# Autodesk Inventor assembly: Assembly1
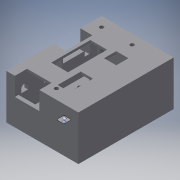
[picture p0: Inventor's stored thumbnail of the model, 180x180]
Saved by Autodesk Inventor 2017 (Build 210142000, 142)
## iProperties
Created: 2017-02-14
Part Number: Assembly1
Document SubType Name: Assembly
Designer: William
Author: William
## Documents named in this file (3)
- F:\Dropbox\Projects\Skateboard\Housing\Assembly1.iam
- F:\Dropbox\Projects\Skateboard\Housing Base.ipt
- F:\Dropbox\Projects\Skateboard\HousingTop.ipt
## Components (2 placed, 2 different names)
1. Housing Base:1 — Mate:1, Flush:1, Flush:2
2. HousingTop:1 — Mate:1, Flush:1, Flush:2
## Relationships (3: Flush 2, Mate 1)
- Mate:1: Housing Base:1 ↔ HousingTop:1
- Flush:1: Housing Base:1 ↔ HousingTop:1
- Flush:2: Housing Base:1 ↔ HousingTop:1
